# Autodesk Inventor assembly: InputJack_Assembly
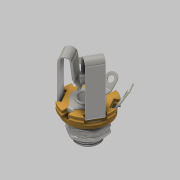
[picture p0: Inventor's stored thumbnail of the model, 180x180]
Saved by Autodesk Inventor 2015 SP1 (Build 190203100, 203)
## iProperties
Created: 2015-06-13
Part Number: InputJack_Assembly
Document SubType Name: Assembly
Designer: Peter Mulkers
Author: Peter Mulkers
## Documents named in this file (8)
- C:\Users\Peter\Documents\InputJack\InputJack_Assembly.iam
- C:\Users\Peter\Documents\InputJack\InputJack_shield.ipt
- C:\Users\Peter\Documents\InputJack\InputJack_partition1.ipt
- C:\Users\Peter\Documents\InputJack\InputJack_partition2.ipt
- C:\Users\Peter\Documents\InputJack\InputJack_nut.ipt
- C:\Users\Peter\Documents\InputJack\InputJack_Washer.ipt
- C:\Users\Peter\Documents\InputJack\InputJack_signal2.ipt
- C:\Users\Peter\Documents\InputJack\InputJack_signal1.ipt
## Components (9 placed, 7 different names)
1. InputJack_shield:1 — Mate:1, Mate:2, Mate:3, Mate:4, Mate:5, Mate:7, Mate:9, Mate:11, Mate:12, Mate:15, Mate:17, Angle:1
2. InputJack_partition1:1 — Mate:1, Mate:2, Mate:13
3. InputJack_partition2:1 — Mate:3, Mate:4, Mate:16
4. InputJack_nut:1 — Mate:5, Mate:8, Mate:11
5. InputJack_Washer:1 — Mate:7, Mate:8, Mate:10
6. InputJack_nut:2 — Mate:9, Mate:10
7. InputJack_partition2:2 — Mate:12, Mate:13, Mate:14
8. InputJack_signal2:1 — Mate:14, Mate:15
9. InputJack_signal1:1 — Mate:16, Mate:17, Angle:1
## Relationships (17: Mate 16, Angle 1)
- Mate:1: InputJack_shield:1 ↔ InputJack_partition1:1
- Mate:2: InputJack_shield:1 ↔ InputJack_partition1:1
- Mate:3: InputJack_shield:1 ↔ InputJack_partition2:1
- Mate:4: InputJack_shield:1 ↔ InputJack_partition2:1
- Mate:5: InputJack_shield:1 ↔ InputJack_nut:1
- Mate:7: InputJack_shield:1 ↔ InputJack_Washer:1
- Mate:8: InputJack_nut:1 ↔ InputJack_Washer:1
- Mate:9: InputJack_shield:1 ↔ InputJack_nut:2
- Mate:10: InputJack_Washer:1 ↔ InputJack_nut:2
- Mate:11: InputJack_shield:1 ↔ InputJack_nut:1
- Mate:12: InputJack_shield:1 ↔ InputJack_partition2:2
- Mate:13: InputJack_partition1:1 ↔ InputJack_partition2:2
- Mate:14: InputJack_partition2:2 ↔ InputJack_signal2:1
- Mate:15: InputJack_shield:1 ↔ InputJack_signal2:1
- Mate:16: InputJack_partition2:1 ↔ InputJack_signal1:1
- Mate:17: InputJack_shield:1 ↔ InputJack_signal1:1
- Angle:1 (60 deg): InputJack_shield:1 ↔ InputJack_signal1:1
